# Autodesk Inventor assembly: Gripper V1.2
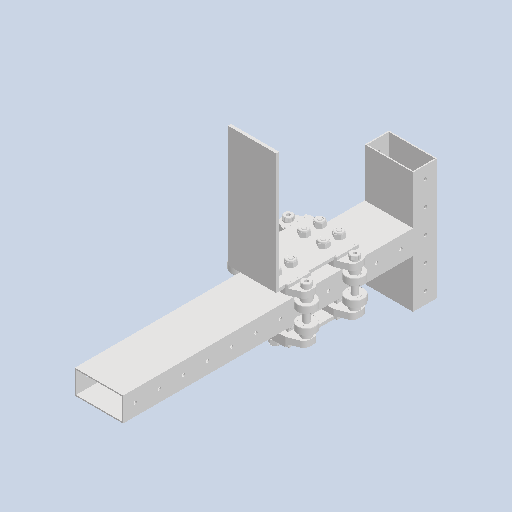
[picture p0: Inventor's stored thumbnail of the model, 512x512]
Saved by Autodesk Inventor 2023 (Build 270158000, 158)
## iProperties
Created: 2023-01-18
Part Number: Gripper V1.2
Document SubType Name: Assembly
Designer: Gabriel - T3 CAD
Author: Gabriel - T3 CAD
## Documents named in this file (7)
- C:\Users\Gabriel - T3 CAD\Documents\GitHub\t3-CAD\T3-CAD\Current Season CAD\Swerve-DriveTrain-V2.1 (LongBot)\Gripper V1.2.iam
- C:\Users\Gabriel - T3 CAD\Documents\GitHub\t3-CAD\T3-CAD\Current Season CAD\Swerve-DriveTrain-V2.1 (LongBot)\Gripper Slider Connecting Plate.ipt
- C:\Users\Gabriel - T3 CAD\Documents\GitHub\t3-CAD\T3-CAD\Stock\ThriftyBot-Elevator\OLD\New folder\Sliding Elevator Block Assembly _1_.iam
- C:\Users\Gabriel - T3 CAD\Documents\GitHub\t3-CAD\T3-CAD\Stock\ThriftyBot-Elevator\OLD\New folder\Sliding Elevator Block Assembly _2_.iam
- C:\Users\Gabriel - T3 CAD\Documents\GitHub\t3-CAD\T3-CAD\Current Season CAD\Swerve-DriveTrain-V2.1 (LongBot)\VersaFrame (Gripper-BaseBar).ipt
- C:\Users\Gabriel - T3 CAD\Documents\GitHub\t3-CAD\T3-CAD\Current Season CAD\Swerve-DriveTrain-V2.1 (LongBot)\VersaFrame (Griper Track Spacer Bar).ipt
- C:\Users\Gabriel - T3 CAD\Documents\GitHub\t3-CAD\T3-CAD\Current Season CAD\Swerve-DriveTrain-V2.1 (LongBot)\Gripper Slider Connecting Plate & Bar.ipt
## Components (8 placed, 6 different names)
1. Sliding Elevator Block Assembly _1_:1 [sub-assembly] — Tangent:2, Tangent:7, Rotational:3, Rotational:4
2. Sliding Elevator Block Assembly _1_:2 [sub-assembly] — Mate:13, Mate:14, Tangent:1, Tangent:5, Rotational:1, Rotational:2, Mate:23
3. Sliding Elevator Block Assembly _2_:1 [sub-assembly] — Mate:7, Mate:9, Mate:10, Mate:13, Mate:14, Tangent:4, Tangent:6, Mate:23
4. Sliding Elevator Block Assembly _2_:2 [sub-assembly] — Mate:8, Mate:11, Mate:12, Tangent:3
5. Gripper Slider Connecting Plate:2 — Mate:7, Mate:8, Mate:9, Mate:10, Mate:11, Mate:12
6. VersaFrame (Gripper-BaseBar):1 — Tangent:1, Tangent:2, Tangent:3, Tangent:4, Tangent:5, Tangent:6, Tangent:7, Mate:20, Mate:21, Mate:22
7. VersaFrame (Griper Track Spacer Bar):1 — Mate:20, Mate:21, Mate:22
8. Gripper Slider Connecting Plate & Bar:1 — Rotational:1, Rotational:2, Rotational:3, Rotational:4
## Relationships (23: Mate 12, Tangent 7, RevoluteJoint 4)
- Mate:7: Sliding Elevator Block Assembly _2_:1 ↔ Gripper Slider Connecting Plate:2
- Mate:8: Sliding Elevator Block Assembly _2_:2 ↔ Gripper Slider Connecting Plate:2
- Mate:9: Sliding Elevator Block Assembly _2_:1 ↔ Gripper Slider Connecting Plate:2
- Mate:10: Sliding Elevator Block Assembly _2_:1 ↔ Gripper Slider Connecting Plate:2
- Mate:11: Sliding Elevator Block Assembly _2_:2 ↔ Gripper Slider Connecting Plate:2
- Mate:12: Sliding Elevator Block Assembly _2_:2 ↔ Gripper Slider Connecting Plate:2
- Mate:13: Sliding Elevator Block Assembly _1_:2 ↔ Sliding Elevator Block Assembly _2_:1
- Mate:14: Sliding Elevator Block Assembly _1_:2 ↔ Sliding Elevator Block Assembly _2_:1
- Tangent:1: Sliding Elevator Block Assembly _1_:2 ↔ VersaFrame (Gripper-BaseBar):1
- Tangent:2: Sliding Elevator Block Assembly _1_:1 ↔ VersaFrame (Gripper-BaseBar):1
- Tangent:3: Sliding Elevator Block Assembly _2_:2 ↔ VersaFrame (Gripper-BaseBar):1
- Tangent:4: Sliding Elevator Block Assembly _2_:1 ↔ VersaFrame (Gripper-BaseBar):1
- Tangent:5: Sliding Elevator Block Assembly _1_:2 ↔ VersaFrame (Gripper-BaseBar):1
- Tangent:6: Sliding Elevator Block Assembly _2_:1 ↔ VersaFrame (Gripper-BaseBar):1
- Tangent:7: Sliding Elevator Block Assembly _1_:1 ↔ VersaFrame (Gripper-BaseBar):1
- Mate:20: VersaFrame (Gripper-BaseBar):1 ↔ VersaFrame (Griper Track Spacer Bar):1
- Mate:21: VersaFrame (Gripper-BaseBar):1 ↔ VersaFrame (Griper Track Spacer Bar):1
- Mate:22 (50.8 mm): VersaFrame (Gripper-BaseBar):1 ↔ VersaFrame (Griper Track Spacer Bar):1
- Rotational:1 [RevoluteJoint]: Sliding Elevator Block Assembly _1_:2 ↔ Gripper Slider Connecting Plate & Bar:1
- Rotational:2 [RevoluteJoint]: Sliding Elevator Block Assembly _1_:2 ↔ Gripper Slider Connecting Plate & Bar:1
- Rotational:3 [RevoluteJoint]: Sliding Elevator Block Assembly _1_:1 ↔ Gripper Slider Connecting Plate & Bar:1
- Rotational:4 [RevoluteJoint]: Sliding Elevator Block Assembly _1_:1 ↔ Gripper Slider Connecting Plate & Bar:1
- Mate:23 (38.354 mm): Sliding Elevator Block Assembly _1_:2 ↔ Sliding Elevator Block Assembly _2_:1
